# Autodesk Inventor assembly: full_assembly
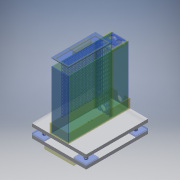
[picture p0: Inventor's stored thumbnail of the model, 180x180]
Saved by Autodesk Inventor 2018.1 (Build 221171000, 171)
## iProperties
Created: 2017-07-30
Part Number: full_assembly
Document SubType Name: Assembly
Designer: Tom
Author: Tom
## Documents named in this file (5)
- \\Mac\Dropbox\2015-2016\Bachelorproef\Inventor\Etstank_v2\full_assembly.iam
- \\Mac\Dropbox\2015-2016\Bachelorproef\Inventor\Etstank_v2\load cell_assembly.iam
- \\Mac\Dropbox\2015-2016\Bachelorproef\Inventor\Etstank_v2\tank_assembly.iam
- \\Mac\Dropbox\2015-2016\Bachelorproef\Inventor\Etstank_v2\surround_assembly.iam
- \\Mac\Dropbox\2015-2016\Bachelorproef\Inventor\Etstank_v2\par.xls
## Components (3 placed, 3 different names)
1. load cell_assembly:1 [sub-assembly] — Mate:1, Flush:1, Flush:2, Mate:2
2. tank_assembly:1 [sub-assembly] — Mate:1, Flush:1, Flush:2, Mate:3, Mate:4
3. surround_assembly:1 [sub-assembly] — Mate:2, Mate:3, Mate:4
## Relationships (6: Mate 4, Flush 2)
- Mate:1: load cell_assembly:1 ↔ tank_assembly:1
- Flush:1 (5.5 mm): load cell_assembly:1 ↔ tank_assembly:1
- Flush:2 (120 mm): load cell_assembly:1 ↔ tank_assembly:1
- Mate:2: load cell_assembly:1 ↔ surround_assembly:1
- Mate:3 (0.5 mm): tank_assembly:1 ↔ surround_assembly:1
- Mate:4 (0.5 mm): tank_assembly:1 ↔ surround_assembly:1
## Named parameters: maxh = 400 mm, maxw = 350 mm, lcsd = 19.05 mm, lcdd = 100 mm, lcwd1 = 25 mm, lcwd2 = 34 mm, lcw = 20 mm, lch1 = 39 mm, lch2 = 40 mm, lcl = 150 mm, lcwd3 = 43 mm, dia1 = 6 mm, td = 18 mm, bhh = 6 mm, bhd = 10 mm, sw = 25 mm, sh = 31 mm, spacert = 2 mm, nutdist = 40 mm, platft = 20 mm, supt = 20 mm, pvct = 5 mm, tankw = 100 mm, tankh = 370 mm, tankl = 379 mm, dia2 = 20 mm, tankv = 1e+07 mm, actual_tankv = 1.4023e+07 mm, dia4 = 11 mm, dia3 = 8 mm, play = 9 mm, holeh = 26 mm, surroundh = 60 mm, slack = 0.5 mm, surroundt = 5 mm, play2 = 3 mm, maxl = 400 mm, diaoverflow = 25 mm, diawater = 25 mm, diaair = 32 mm, diaph = 32 mm, extra_height = 100 mm, diacucl = 32 mm, mindist = 80 mm, distfromedge = 10 mm, diasurroundhole = 42 mm, sensorsupportl = 100 mm, diagrate = 12 mm, brachetw = 10 mm, gratespacing = 12.02082 mm, sidedist = 13.9375 mm, bottomdist = 9.6355 mm, diahcl = 32 mm, diafloat = 50 mm, bracketw = 10 mm, bracketwtop = 6 mm, bracketwbottom = 6 mm, handlew = 50 mm, handlel = 120 mm, handlesupporth = 20 mm, nett = 1 mm, nethole = 16 mm, netside = 3.5 mm, nettop = 7 mm, netholespacing = 2 mm, nutholdert = 10 mm, diaetape = 32 mm
